# Autodesk Inventor assembly: Coins inferieur
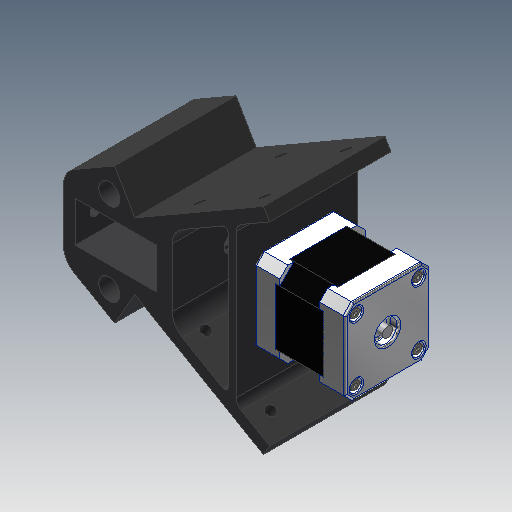
[picture p0: Inventor's stored thumbnail of the model, 512x512]
Saved by Autodesk Inventor 2017 (Build 210142000, 142)
## iProperties
Part Number: Coins inferieur
Material: Générique
Document SubType Name: Assembly
Mass: 642.317 g
Surface Area: 748.928 cm^2
Volume: 235.036 cm^3
Density: 2.73284 g/cm^3
Stock Number: 1420-01-14
Project: 1420 Vauban 3D XL
## Documents named in this file (6)
- W:\Professionnel\Conception FABLAB\1420-Vauban 3D XL\1420-01 Armature\1420-01-14 Coins inferieur.iam
- W:\Professionnel\Conception FABLAB\1420-Vauban 3D XL\1420-01 Armature\1420-01-05 Coins inferieur.ipt
- W:\Professionnel\Conception FABLAB\1420-Vauban 3D XL\1420-11 Electronique\1420-11-01  Nema 17\1420-11-40 Nema 17.iam
- W:\Professionnel\Conception FABLAB\1420-Vauban 3D XL\1420-01 Armature\1420-01-10 Poulie.ipt
- W:\Professionnel\Conception FABLAB\1420-Vauban 3D XL\1420-90 Centre de contenu\fr-FR\DIN 125-1  A\DIN 125 - A 3,2.ipt
- W:\Professionnel\Conception FABLAB\1420-Vauban 3D XL\1420-90 Centre de contenu\fr-FR\ANSI B18.3.1M(1)\ANSI B18.3.1M - M3x0,5 x 10(2).ipt
## Components (11 placed, 5 different names)
1. 1420-01-05 Coins inferieur:1 — Placage:1, Placage:2, Placage:3, Placage:5, Placage:7, Placage:8, Placage:9, Placage:10, Placage:11, Placage:12, Placage:13, Placage:15
2. 1420-11-40 Nema 17:1 [sub-assembly] — Placage:1, Placage:2, Placage:3, Placage:6
3. 1420-01-10 Poulie:1 — Placage:5, Placage:6
4. DIN 125-1 A A 3,2:1 — Affleurement:3, Placage:10, Placage:14
5. DIN 125-1 A A 3,2:2 — Affleurement:2, Affleurement:3, Placage:11
6. DIN 125-1 A A 3,2:3 — Affleurement:1, Placage:7, Placage:8
7. DIN 125-1 A A 3,2:4 — Affleurement:1, Affleurement:2, Placage:9, Placage:16
8. Vis à tête percée - Métrique M3x0,5 x 10:1 — Affleurement:4, Placage:12
9. Vis à tête percée - Métrique M3x0,5 x 10:2 — Affleurement:4, Affleurement:5, Placage:13, Placage:16
10. Vis à tête percée - Métrique M3x0,5 x 10:3 — Affleurement:5, Affleurement:6, Placage:14
11. Vis à tête percée - Métrique M3x0,5 x 10:4 — Affleurement:6, Placage:15
## Relationships (21: Mate 15, Flush 6)
- Placage:1 [Mate]: 1420-01-05 Coins inferieur:1 ↔ 1420-11-40 Nema 17:1
- Placage:2 [Mate]: 1420-01-05 Coins inferieur:1 ↔ 1420-11-40 Nema 17:1
- Placage:3 [Mate]: 1420-01-05 Coins inferieur:1 ↔ 1420-11-40 Nema 17:1
- Placage:5 [Mate] (3.5 mm): 1420-01-05 Coins inferieur:1 ↔ 1420-01-10 Poulie:1
- Placage:6 [Mate]: 1420-11-40 Nema 17:1 ↔ 1420-01-10 Poulie:1
- Affleurement:1 [Flush]: DIN 125-1 A A 3,2:3 ↔ DIN 125-1 A A 3,2:4
- Affleurement:2 [Flush]: DIN 125-1 A A 3,2:2 ↔ DIN 125-1 A A 3,2:4
- Affleurement:3 [Flush]: DIN 125-1 A A 3,2:1 ↔ DIN 125-1 A A 3,2:2
- Placage:7 [Mate]: 1420-01-05 Coins inferieur:1 ↔ DIN 125-1 A A 3,2:3
- Placage:8 [Mate]: 1420-01-05 Coins inferieur:1 ↔ DIN 125-1 A A 3,2:3
- Placage:9 [Mate]: 1420-01-05 Coins inferieur:1 ↔ DIN 125-1 A A 3,2:4
- Placage:10 [Mate]: 1420-01-05 Coins inferieur:1 ↔ DIN 125-1 A A 3,2:1
- Placage:11 [Mate]: 1420-01-05 Coins inferieur:1 ↔ DIN 125-1 A A 3,2:2
- Affleurement:4 [Flush]: Vis à tête percée - Métrique M3x0,5 x 10:1 ↔ Vis à tête percée - Métrique M3x0,5 x 10:2
- Affleurement:5 [Flush]: Vis à tête percée - Métrique M3x0,5 x 10:2 ↔ Vis à tête percée - Métrique M3x0,5 x 10:3
- Affleurement:6 [Flush]: Vis à tête percée - Métrique M3x0,5 x 10:3 ↔ Vis à tête percée - Métrique M3x0,5 x 10:4
- Placage:12 [Mate]: 1420-01-05 Coins inferieur:1 ↔ Vis à tête percée - Métrique M3x0,5 x 10:1
- Placage:13 [Mate]: 1420-01-05 Coins inferieur:1 ↔ Vis à tête percée - Métrique M3x0,5 x 10:2
- Placage:14 [Mate]: DIN 125-1 A A 3,2:1 ↔ Vis à tête percée - Métrique M3x0,5 x 10:3
- Placage:15 [Mate]: 1420-01-05 Coins inferieur:1 ↔ Vis à tête percée - Métrique M3x0,5 x 10:4
- Placage:16 [Mate]: DIN 125-1 A A 3,2:4 ↔ Vis à tête percée - Métrique M3x0,5 x 10:2
